# Autodesk Inventor assembly: gripper-adapter-as
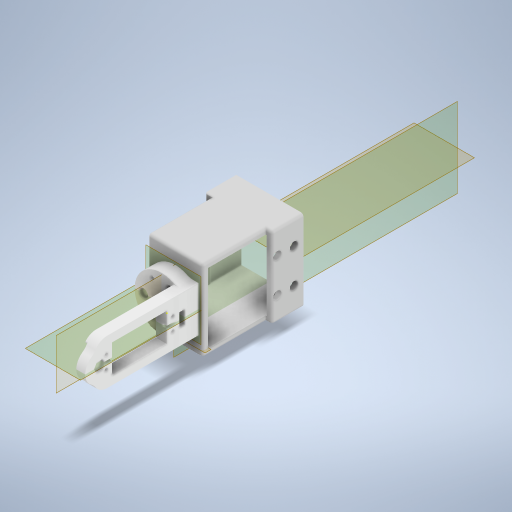
[picture p0: Inventor's stored thumbnail of the model, 512x512]
Saved by Autodesk Inventor 2024 (Build 280153000, 153)
## iProperties
Created: 2024-04-26
Part Number: gripper-adapter-as
Document SubType Name: Assembly
Designer: MaartenGeorgesBuelen
Author: MaartenGeorgesBuelen
## Documents named in this file (4)
- C:\Users\MaartenGeorgesBuelen\Documents\Inventor\robot arm\gripper-adapter-as.iam
- C:\Users\MaartenGeorgesBuelen\Documents\Inventor\robot arm\upper arm.ipt
- C:\Users\MaartenGeorgesBuelen\Documents\Inventor\robot arm\other gripper\ServoMount.ipt
- C:\Users\MaartenGeorgesBuelen\Documents\Inventor\robot arm\gripper-adapter.ipt
## Components (3 placed, 3 different names)
1. upper arm:1 — Mate:3, Mate:5, Mate:6, Mate:7, Angle:1, Angle:2, Mate:9, Flush:4, Flush:5
2. ServoMount:1 — Mate:5, Mate:6, Mate:7, Flush:1
3. gripper-adapter:1 — Flush:1, Mate:9, Flush:4, Flush:5
## Relationships (10: Mate 5, Flush 3, Angle 2)
- Mate:3: upper arm:1
- Mate:5 (30 mm): upper arm:1 ↔ ServoMount:1
- Mate:6: upper arm:1 ↔ ServoMount:1
- Mate:7: upper arm:1 ↔ ServoMount:1
- Angle:1 (90 deg): upper arm:1
- Angle:2 (0 deg): upper arm:1
- Flush:1: ServoMount:1 ↔ gripper-adapter:1
- Mate:9: upper arm:1 ↔ gripper-adapter:1
- Flush:4: upper arm:1 ↔ gripper-adapter:1
- Flush:5: upper arm:1 ↔ gripper-adapter:1
